# Autodesk Inventor assembly: Room_Complete_Assembly
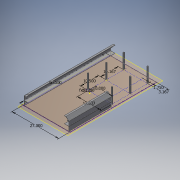
[picture p0: Inventor's stored thumbnail of the model, 180x180]
Saved by Autodesk Inventor 2019 (Build 230136000, 136)
## iProperties
Created: 2020-10-31
Part Number: Room_Complete_Assembly
Document SubType Name: Assembly
Designer: close
Author: close
## Documents named in this file (3)
- C:\Users\close\Desktop\BARC-ROAR\barc_hardware\RFS B0164 Indoor CAD\Room_Complete_Assembly.iam
- C:\Users\close\Desktop\BARC-ROAR\barc_hardware\RFS B0164 Indoor CAD\ROOM_B164.ipt
- C:\Users\close\Desktop\BARC-ROAR\barc_hardware\RFS B0164 Indoor CAD\Platform_1.ipt
## Components (2 placed, 2 different names)
1. ROOM_B164:1 — Mate:1, Flush:1, Flush:2
2. Platform_1:1 — Flush:1, Flush:2
## Relationships (3: Flush 2, Mate 1)
- Mate:1: ROOM_B164:1
- Flush:1: ROOM_B164:1 ↔ Platform_1:1
- Flush:2: ROOM_B164:1 ↔ Platform_1:1
